# Autodesk Inventor assembly: Wine Rack and Light Shelf Assembly
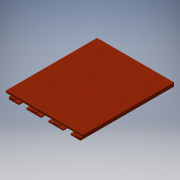
[picture p0: Inventor's stored thumbnail of the model, 180x180]
Saved by Autodesk Inventor 2016 (Build 200138000, 138)
## iProperties
Created: 2017-11-04
Part Number: Wine Rack and Light Shelf Assembly
Document SubType Name: Assembly
Designer: mathaetaes
Author: mathaetaes
## Documents named in this file (4)
- E:\Projects\3D Printer\printer projects\My Designs\Bar Cabinet 2.2.2018\Wine Rack and Light Shelf Assembly Right.iam
- E:\Projects\3D Printer\printer projects\My Designs\Bar Cabinet 2.2.2018\Horizontal Shelf with Lights.ipt
- E:\Projects\3D Printer\printer projects\My Designs\Bar Cabinet 2.2.2018\Wine Glass Rack Full Assembly.iam
- E:\Projects\3D Printer\printer projects\My Designs\Bar Cabinet 2.2.2018\LED light strip.ipt
## Components (5 placed, 3 different names)
1. Horizontal Shelf with Lights:1 — Mate:1, Flush:5, Mate:5, Mate:6, Mate:7, Flush:6
2. Wine Glass Rack Full Assembly:1 [sub-assembly] — Mate:1, Flush:5, Flush:6
3. LED light strip:4 — Mate:5
4. LED light strip:5 — Mate:6
5. LED light strip:6 — Mate:7
## Relationships (6: Mate 4, Flush 2)
- Mate:1: Horizontal Shelf with Lights:1 ↔ Wine Glass Rack Full Assembly:1
- Flush:5 (-12.7 mm): Horizontal Shelf with Lights:1 ↔ Wine Glass Rack Full Assembly:1
- Mate:5: Horizontal Shelf with Lights:1 ↔ LED light strip:4
- Mate:6: Horizontal Shelf with Lights:1 ↔ LED light strip:5
- Mate:7: Horizontal Shelf with Lights:1 ↔ LED light strip:6
- Flush:6: Horizontal Shelf with Lights:1 ↔ Wine Glass Rack Full Assembly:1
